# Autodesk Inventor assembly: Arm_MiniLink_9
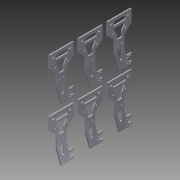
[picture p0: Inventor's stored thumbnail of the model, 180x180]
Saved by Autodesk Inventor 2013 (Build 170138000, 138)
## iProperties
Created: 2014-05-18
Part Number: Arm_MiniLink_9
Document SubType Name: Assembly
Designer: andou
Author: andou
## Documents named in this file (2)
- C:\Users\andou\Documents\Inventor\RoboticsProject\project_4\Robot\Arm\Arm_MiniLink_6.iam
- C:\Users\andou\Documents\Inventor\RoboticsProject\project_4\Robot\Arm\Arm_MiniLink.ipt
## Components (6 placed, 1 different names)
1. Arm_MiniLink:1
2. Arm_MiniLink:2
3. Arm_MiniLink:3
4. Arm_MiniLink:4
5. Arm_MiniLink:5
6. Arm_MiniLink:6
## Component patterns: (6 elements, first: Arm_MiniLink:1)
